# Autodesk Inventor assembly: Frame
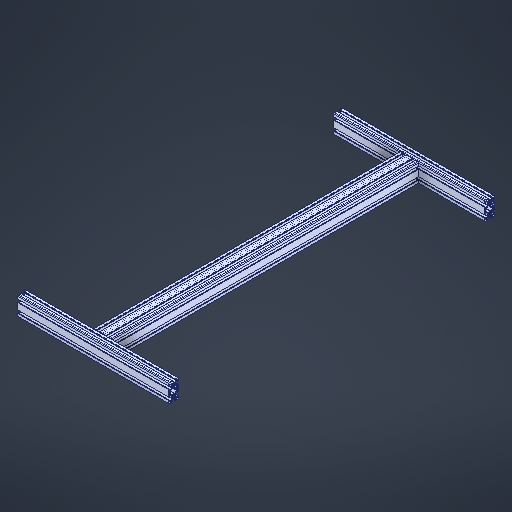
[picture p0: Inventor's stored thumbnail of the model, 512x512]
Saved by Autodesk Inventor 2025 (Build 290162000, 162)
## iProperties
Created: 2025-05-16
Part Number: Frame
Document SubType Name: Assembly
Designer: mayhe
Author: mayhe
## Documents named in this file (3)
- C:\Users\mayhe\OneDrive\Documents\GitHub\In-situ-monitoring-of-powder-bed-fusion-additive-manufacturing\system_development\Orichalcum\v0.2\Hardware_design\custom-cover\Frame.iam
- C:\Users\mayhe\Downloads\AL11604-NONSEALED\8020-20-4040 X 0_65 M\8020-20-4040 X 0_65 M.ipt
- C:\Users\mayhe\OneDrive\Documents\GitHub\In-situ-monitoring-of-powder-bed-fusion-additive-manufacturing\system_development\Orichalcum\v0.2\Hardware_design\custom-cover\Frame 8080s\8020-20-2040 X 0_32 M\8020-20-.ipt
## Components (3 placed, 2 different names)
1. 8020-20-4040 X 0_65 M:1 — Mate:1, Flush:1, Flush:2, Mate:2, Flush:3, Flush:4
2. 8020-20-:1 — Mate:1, Flush:1, Flush:2
3. 8020-20-:2 — Mate:2, Flush:3, Flush:4
## Relationships (6: Flush 4, Mate 2)
- Mate:1: 8020-20-4040 X 0_65 M:1 ↔ 8020-20-:1
- Flush:1: 8020-20-4040 X 0_65 M:1 ↔ 8020-20-:1
- Flush:2 (-140 mm): 8020-20-4040 X 0_65 M:1 ↔ 8020-20-:1
- Mate:2: 8020-20-4040 X 0_65 M:1 ↔ 8020-20-:2
- Flush:3: 8020-20-4040 X 0_65 M:1 ↔ 8020-20-:2
- Flush:4 (-140 mm): 8020-20-4040 X 0_65 M:1 ↔ 8020-20-:2
